# Autodesk Inventor assembly: ArcadeController
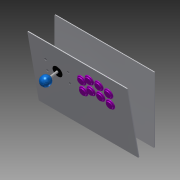
[picture p0: Inventor's stored thumbnail of the model, 180x180]
Saved by Autodesk Inventor 2013 (Build 170138000, 138)
## iProperties
Created: 2013-01-27
Part Number: ArcadeController
Document SubType Name: Assembly
Designer: xylzlyx
Author: xylzlyx
## Documents named in this file (8)
- C:\dev\pewpew\assemblies\ArcadeController.iam
- C:\dev\pewpew\parts\Panel_bottom.ipt
- C:\dev\pewpew\parts\Panel_top.ipt
- C:\dev\pewpew\parts\JLF-TP-8YT_ball.ipt
- C:\dev\pewpew\parts\JLF-TP-8YT_body.ipt
- C:\dev\pewpew\parts\JLF-TP-8YT_ring.ipt
- C:\dev\pewpew\assemblies\ArcadeController\Design Accelerator\Bolted Connection2.iam
- C:\dev\pewpew\parts\OBSF-30-B_button.ipt
## Components (14 placed, 7 different names)
1. BottomPanel:1 — Mate:1, Flush:1, Flush:2, Flush:3, Angle:1
2. TopPanel:1 — Flush:1, Flush:2, Flush:3, Insert:1, Mate:4, Mate:5, Insert:4, Insert:5, Insert:6, Insert:7, Insert:8, Insert:9, Insert:10, Insert:11, Angle:1
3. JoystickBall:1 — Insert:2
4. JoystickBody:1 — Insert:1, Insert:2, Insert:3
5. JoystickCover:1 — Insert:3
6. Bolted Connection:1 [sub-assembly] — Mate:4, Mate:5
7. OBSF-30-B_button:1 — Insert:4
8. OBSF-30-B_button:2 — Insert:5
9. OBSF-30-B_button:3 — Insert:6
10. OBSF-30-B_button:4 — Insert:7
11. OBSF-30-B_button:5 — Insert:8
12. OBSF-30-B_button:6 — Insert:9
13. OBSF-30-B_button:7 — Insert:10
14. OBSF-30-B_button:8 — Insert:11
## Relationships (18: Insert 11, Mate 3, Flush 3, Angle 1)
- Mate:1: BottomPanel:1
- Flush:1: BottomPanel:1 ↔ TopPanel:1
- Flush:2: BottomPanel:1 ↔ TopPanel:1
- Flush:3: BottomPanel:1 ↔ TopPanel:1
- Insert:1: TopPanel:1 ↔ JoystickBody:1
- Insert:2: JoystickBall:1 ↔ JoystickBody:1
- Mate:4: TopPanel:1 ↔ Bolted Connection:1
- Mate:5: TopPanel:1 ↔ Bolted Connection:1
- Insert:3 (3 mm): JoystickBody:1 ↔ JoystickCover:1
- Insert:4: TopPanel:1 ↔ OBSF-30-B_button:1
- Insert:5: TopPanel:1 ↔ OBSF-30-B_button:2
- Insert:6: TopPanel:1 ↔ OBSF-30-B_button:3
- Insert:7: TopPanel:1 ↔ OBSF-30-B_button:4
- Insert:8: TopPanel:1 ↔ OBSF-30-B_button:5
- Insert:9: TopPanel:1 ↔ OBSF-30-B_button:6
- Insert:10: TopPanel:1 ↔ OBSF-30-B_button:7
- Insert:11: TopPanel:1 ↔ OBSF-30-B_button:8
- Angle:1 (190 deg): BottomPanel:1 ↔ TopPanel:1
